# Autodesk Inventor assembly: 144x9
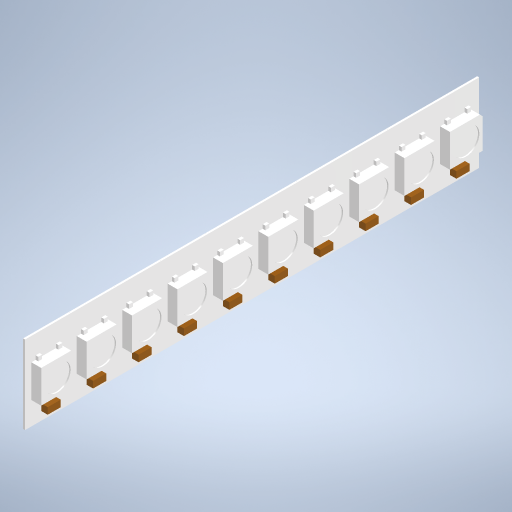
[picture p0: Inventor's stored thumbnail of the model, 512x512]
Saved by Autodesk Inventor 2023 (Build 270158000, 158)
## iProperties
Created: 2024-03-20
Part Number: 144x9
Document SubType Name: Assembly
Designer: noname
Author: noname
## Documents named in this file (2)
- C:\Users\noname\Documents\GitHub\AudMix\3dModels\LedStrip\144x9.iam
- C:\Users\noname\Documents\GitHub\AudMix\3dModels\LedStrip\Base144.ipt
## Components (10 placed, 1 different names)
1. Base144:1
2. Base144:2
3. Base144:3
4. Base144:4
5. Base144:5
6. Base144:6
7. Base144:7
8. Base144:8
9. Base144:9
10. Base144:10
## Component patterns: (10 elements, first: Base144:1)
